# Autodesk Inventor assembly: RoboCupHumanoidLeagueSoccerField_KidSize
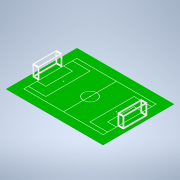
[picture p0: Inventor's stored thumbnail of the model, 180x180]
Saved by Autodesk Inventor 2022 (Build 260153000, 153)
## iProperties
Created: 2022-10-30
Part Number: RoboCupHumanoidLeagueSoccerField_KidSize
Document SubType Name: Assembly
Designer: Masato Kubotera
Author: Masato Kubotera
## Documents named in this file (3)
- C:\Users\MasatoKubotera\Desktop\RoboCupHumanoidLeagueSoccerField_KidSize.iam
- C:\Users\MasatoKubotera\Desktop\Goal.ipt
- C:\Users\MasatoKubotera\Desktop\RoboCupHumanoidLeagueSoccerField_KidSize.ipt
## Components (3 placed, 2 different names)
1. RoboCupHumanoidLeagueSoccerField_KidSize:1 — フラッシュ:1, フラッシュ:2, フラッシュ:3, フラッシュ:4, フラッシュ:5, メイト:1
2. Goal:1 — フラッシュ:4, フラッシュ:5, メイト:1
3. Goal:2
## Relationships (6: Flush 5, Mate 1)
- フラッシュ:1 [Flush]: RoboCupHumanoidLeagueSoccerField_KidSize:1
- フラッシュ:2 [Flush]: RoboCupHumanoidLeagueSoccerField_KidSize:1
- フラッシュ:3 [Flush]: RoboCupHumanoidLeagueSoccerField_KidSize:1
- フラッシュ:4 [Flush]: RoboCupHumanoidLeagueSoccerField_KidSize:1 ↔ Goal:1
- フラッシュ:5 [Flush]: RoboCupHumanoidLeagueSoccerField_KidSize:1 ↔ Goal:1
- メイト:1 [Mate]: RoboCupHumanoidLeagueSoccerField_KidSize:1 ↔ Goal:1
